# Autodesk Inventor assembly: assembly profil masca
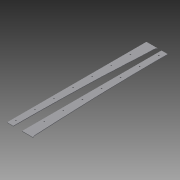
[picture p0: Inventor's stored thumbnail of the model, 180x180]
Saved by Autodesk Inventor 2015 SP1 (Build 190203100, 203)
## iProperties
Created: 2015-10-21
Part Number: assembly profil masca
Document SubType Name: Assembly
Designer: ubik
Author: ubik
## Documents named in this file (3)
- C:\Users\ubik\Dropbox\DueTech\webasto\assembly profil masca.iam
- C:\Users\ubik\Dropbox\DueTech\webasto\profil masca dreapta.ipt
- C:\Users\ubik\Dropbox\DueTech\webasto\profil masca 1.ipt
## Components (2 placed, 2 different names)
1. profil masca 1:1 — Flush:1, Flush:2
2. profil masca dreapta:1 — Flush:1, Flush:2
## Relationships (2: Flush 2)
- Flush:1: profil masca 1:1 ↔ profil masca dreapta:1
- Flush:2: profil masca 1:1 ↔ profil masca dreapta:1
